# Autodesk Inventor assembly: 24813005
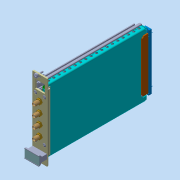
[picture p0: Inventor's stored thumbnail of the model, 180x180]
Saved by Autodesk Inventor 2016 (Build 200138000, 138)
## iProperties
Company: TraceParts S.A.
Created: 2016-05-18
Part Number: 24813005
Checked By: TraceParts S.A.
Catalog Web Link: www.traceparts.com
Vendor: Pentair/Schroff
Document SubType Name: Assembly
Designer: TraceParts
REFERENCE: 24813005
SUPPLIER: Pentair/Schroff
TraceParts.PartNumber: 30-07022014-094149
TraceParts.PartTitle: Frame-type plug-in units PRO with hood, 3 U, front panel shielded (textile gasket)
TraceParts.InstanceId: 30-07022014-0941498DKL5QO617MFTN2NAWYE3DVT9
TraceParts.PartStatus: Published
TraceParts.PartVersion: 1.0.8
TRACEPARTS: TRACEPARTS
TraceParts.PartLanguage: en
TraceParts.ClassPath: SCHROFF:/F_SCHROFF/SCHROFF.8/SCHROFF.8.2/SCHROFF.8.2.1/30-07022014-094149
Author: TraceParts
## Documents named in this file (30)
- C:\Users\Zara\Documents\hera-cad\Node\PAMmodule\24813005.iam
- C:\Users\Zara\Documents\hera-cad\Node\PAMmodule\24813005_28.ipt
- C:\Users\Zara\Documents\hera-cad\Node\PAMmodule\24813005_27.ipt
- C:\Users\Zara\Documents\hera-cad\Node\PAMmodule\24813005_26.ipt
- C:\Users\Zara\Documents\hera-cad\Node\PAMmodule\24813005_25.ipt
- C:\Users\Zara\Documents\hera-cad\Node\PAMmodule\24813005_24.ipt
- C:\Users\Zara\Documents\hera-cad\Node\PAMmodule\24813005_23.ipt
- C:\Users\Zara\Documents\hera-cad\Node\PAMmodule\24813005_22.ipt
- C:\Users\Zara\Documents\hera-cad\Node\PAMmodule\24813005_21.ipt
- C:\Users\Zara\Documents\hera-cad\Node\PAMmodule\24813005_20.ipt
- C:\Users\Zara\Documents\hera-cad\Node\PAMmodule\24813005_19.ipt
- C:\Users\Zara\Documents\hera-cad\Node\PAMmodule\24813005_18.ipt
- C:\Users\Zara\Documents\hera-cad\Node\PAMmodule\24813005_17.ipt
- C:\Users\Zara\Documents\hera-cad\Node\PAMmodule\24813005_16.ipt
- C:\Users\Zara\Documents\hera-cad\Node\PAMmodule\24813005_15.ipt
- C:\Users\Zara\Documents\hera-cad\Node\PAMmodule\24813005_14.ipt
- C:\Users\Zara\Documents\hera-cad\Node\PAMmodule\24813005_13.ipt
- C:\Users\Zara\Documents\hera-cad\Node\PAMmodule\24813005_12.ipt
- C:\Users\Zara\Documents\hera-cad\Node\PAMmodule\24813005_11.ipt
- C:\Users\Zara\Documents\hera-cad\Node\PAMmodule\24813005_10.ipt
- C:\Users\Zara\Documents\hera-cad\Node\PAMmodule\24813005_09.ipt
- C:\Users\Zara\Documents\hera-cad\Node\PAMmodule\24813005_08.ipt
- C:\Users\Zara\Documents\hera-cad\Node\PAMmodule\24813005_07.ipt
- C:\Users\Zara\Documents\hera-cad\Node\PAMmodule\24813005_06.ipt
- C:\Users\Zara\Documents\hera-cad\Node\PAMmodule\24813005_05.ipt
- C:\Users\Zara\Documents\hera-cad\Node\PAMmodule\24813005_04.ipt
- C:\Users\Zara\Documents\hera-cad\Node\PAMmodule\24813005_03.ipt
- C:\Users\Zara\Documents\hera-cad\Node\PAMmodule\24813005_02.ipt
- C:\Users\Zara\Documents\hera-cad\Node\PAMmodule\24813005_01.ipt
- C:\Users\Zara\Documents\hera-cad\Node\SMA Jack Bulkhead small nut.ipt
## Components (32 placed, 29 different names)
1. 24813005_28:1
2. 24813005_27:1
3. 24813005_26:1
4. 24813005_25:1
5. 24813005_24:1
6. 24813005_23:1 — Flush:1, Mate:1, Flush:2, Mate:2, Flush:3, Mate:3, Flush:4, Mate:4
7. 24813005_22:1
8. 24813005_21:1
9. 24813005_20:1
10. 24813005_19:1
11. 24813005_18:1
12. 24813005_17:1
13. 24813005_16:1
14. 24813005_15:1
15. 24813005_14:1
16. 24813005_13:1
17. 24813005_12:1
18. 24813005_11:1
19. 24813005_10:1
20. 24813005_09:1
21. 24813005_08:1
22. 24813005_07:1
23. 24813005_06:1
24. 24813005_05:1
25. 24813005_04:1
26. 24813005_03:1
27. 24813005_02:1
28. 24813005_01:1
29. SMA Jack Bulkhead small nut:1 — Flush:1, Mate:1
30. SMA Jack Bulkhead small nut:2 — Flush:4, Mate:4
31. SMA Jack Bulkhead small nut:3 — Flush:2, Mate:2
32. SMA Jack Bulkhead small nut:4 — Flush:3, Mate:3
## Relationships (8: Flush 4, Mate 4)
- Flush:1: 24813005_23:1 ↔ SMA Jack Bulkhead small nut:1
- Mate:1: 24813005_23:1 ↔ SMA Jack Bulkhead small nut:1
- Flush:2: 24813005_23:1 ↔ SMA Jack Bulkhead small nut:3
- Mate:2: 24813005_23:1 ↔ SMA Jack Bulkhead small nut:3
- Flush:3: 24813005_23:1 ↔ SMA Jack Bulkhead small nut:4
- Mate:3: 24813005_23:1 ↔ SMA Jack Bulkhead small nut:4
- Flush:4: 24813005_23:1 ↔ SMA Jack Bulkhead small nut:2
- Mate:4: 24813005_23:1 ↔ SMA Jack Bulkhead small nut:2
